# Autodesk Inventor assembly: タミヤダンパーフロント56,74.5_MIR
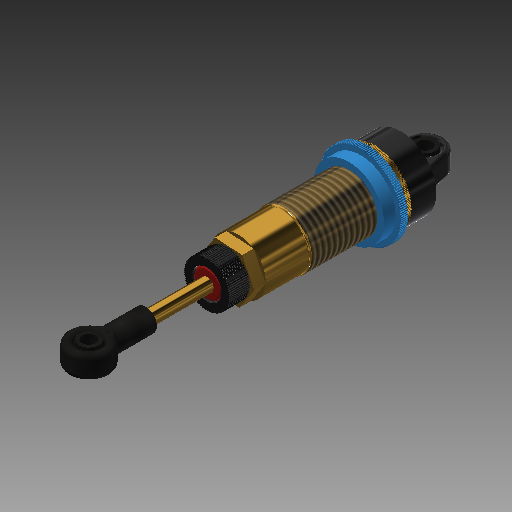
[picture p0: Inventor's stored thumbnail of the model, 512x512]
Saved by Autodesk Inventor 2019.2 (Build 232265000, 265)
## iProperties
Part Number: タミヤダンパーフロント56,74.5_MIR
Material: 一般
Document SubType Name: Assembly
Designer: 雪村
Mass: 29.979 g
Surface Area: 59.981 cm^2
Volume: 5.28585 cm^3
Density: 5.67156 g/cm^3
Author: 雪村
## Documents named in this file (9)
- C:\Users\white\Documents\SRDC\SRDC\Inventor_2017\2018年機体\パーツ\タミヤダンパーフロント56,74.5_MIR.iam
- C:\Users\white\Documents\SRDC\SRDC\Inventor_2017\2018年機体\パーツ\タミヤダンパー1_MIR.ipt
- C:\Users\white\Documents\SRDC\SRDC\Inventor_2017\2018年機体\パーツ\タミヤダンパー2_MIR1.ipt
- C:\Users\white\Documents\SRDC\SRDC\Inventor_2017\2018年機体\パーツ\タミヤダンパー3_MIR1.ipt
- C:\Users\white\Documents\SRDC\SRDC\Inventor_2017\2018年機体\パーツ\タミヤダンパー4_MIR1.ipt
- C:\Users\white\Documents\SRDC\SRDC\Inventor_2017\2018年機体\パーツ\タミヤダンパー6_MIR2.ipt
- C:\Users\white\Documents\SRDC\SRDC\Inventor_2017\2018年機体\パーツ\タミヤダンパー5_MIR1.ipt
- C:\Users\white\Documents\SRDC\SRDC\Inventor_2017\2018年機体\パーツ\タミヤダンパー7_MIR1.ipt
- C:\Users\white\Documents\SRDC\SRDC\Inventor_2017\2018年機体\パーツ\タミヤダンパー8_MIR1.ipt
## Components (9 placed, 8 different names)
1. タミヤダンパー1_MIR:1 — 挿入:1, フラッシュ:1, フラッシュ:3, ボール:2
2. タミヤダンパー2_MIR1:1 — 挿入:1, 挿入:4, メイト:1
3. タミヤダンパー3_MIR1:1 — 挿入:4, 挿入:3
4. タミヤダンパー4_MIR1:1 — メイト:1
5. タミヤダンパー6_MIR2:1 — 挿入:3
6. タミヤダンパー5_MIR1:1 — 挿入:5
7. タミヤダンパー7_MIR1:1 — 挿入:5, フラッシュ:1
8. タミヤダンパー8_MIR1:1 — フラッシュ:3, フラッシュ:2, ボール:2
9. タミヤダンパー8_MIR1:2 — フラッシュ:2
## Relationships (9: Insert 4, Flush 3, Mate 1, BallJoint 1)
- 挿入:1 [Insert]: タミヤダンパー1_MIR:1 ↔ タミヤダンパー2_MIR1:1
- 挿入:4 [Insert]: タミヤダンパー2_MIR1:1 ↔ タミヤダンパー3_MIR1:1
- メイト:1 [Mate]: タミヤダンパー2_MIR1:1 ↔ タミヤダンパー4_MIR1:1
- 挿入:3 [Insert]: タミヤダンパー3_MIR1:1 ↔ タミヤダンパー6_MIR2:1
- 挿入:5 [Insert]: タミヤダンパー5_MIR1:1 ↔ タミヤダンパー7_MIR1:1
- フラッシュ:1 [Flush]: タミヤダンパー1_MIR:1 ↔ タミヤダンパー7_MIR1:1
- フラッシュ:3 [Flush]: タミヤダンパー1_MIR:1 ↔ タミヤダンパー8_MIR1:1
- フラッシュ:2 [Flush]: タミヤダンパー8_MIR1:1 ↔ タミヤダンパー8_MIR1:2
- ボール:2 [BallJoint]: タミヤダンパー1_MIR:1 ↔ タミヤダンパー8_MIR1:1
